# Autodesk Inventor assembly: Z assembly
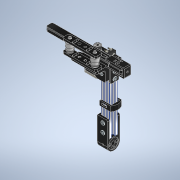
[picture p0: Inventor's stored thumbnail of the model, 180x180]
Saved by Autodesk Inventor 2022 (Build 260153000, 153)
## iProperties
Created: 2022-03-06
Part Number: Z assembly
Document SubType Name: Assembly
Designer: JK
Author: JK
## Documents named in this file (28)
- C:\Users\JK\Documents\Inventor\ScaraNema\SCARA-3DP\Parts\Forearm\Forearm assembly.iam
- C:\Users\JK\Documents\Inventor\ScaraNema\SCARA-3DP\Parts\Forearm\Z Motor support.ipt
- C:\Users\JK\Documents\Inventor\ScaraNema\SCARA-3DP\Parts\V-Slot 20x20.ipt
- C:\Users\JK\Documents\Inventor\ScaraNema\SCARA-3DP\Parts\Forearm\Z axis limit switch support.ipt
- C:\Users\JK\Documents\Inventor\ScaraNema\SCARA-3DP\Parts\Common components\V-Slot 20x20\V-Slot 20x20x150.ipt
- C:\Users\JK\Documents\Inventor\ScaraNema\SCARA-3DP\Parts\Forearm\Forearm support.ipt
- C:\Users\JK\Documents\Inventor\ScaraNema\SCARA-3DP\Parts\Common components\Limit switch.ipt
- C:\Users\JK\Documents\Inventor\ScaraNema\SCARA-3DP\Parts\Fasteners\M2x10 socket bolt.ipt
- C:\Users\JK\Documents\Inventor\ScaraNema\SCARA-3DP\Parts\Fasteners\M2 Hex nut.ipt
- C:\Users\JK\Documents\Inventor\ScaraNema\SCARA-3DP\Parts\Fasteners\M3x10 set screw.ipt
- C:\Users\JK\Documents\Inventor\ScaraNema\SCARA-3DP\Parts\Fasteners\M5x15 Flat head bolt.ipt
- C:\Users\JK\Documents\Inventor\ScaraNema\SCARA-3DP\Parts\Fasteners\M5x10 Flat head bolt.ipt
- C:\Users\JK\Documents\Inventor\ScaraNema\SCARA-3DP\Parts\Fasteners\M5x8 Flat head bolt.ipt
- C:\Users\JK\Documents\Inventor\ScaraNema\SCARA-3DP\Parts\Fasteners\M3 Hex nut.ipt
- C:\Users\JK\Documents\Inventor\ScaraNema\SCARA-3DP\Parts\Fasteners\M5 T-Nut Drop-in 20x20.ipt
- C:\Users\JK\Documents\Inventor\ScaraNema\SCARA-3DP\Parts\Fasteners\M3x6 socket bolt.ipt
- C:\Users\JK\Documents\Inventor\ScaraNema\SCARA-3DP\Parts\Forearm\yystop.ipt
- C:\Users\JK\Documents\Inventor\ScaraNema\SCARA-3DP\Parts\Forearm\Nema14 Stepper Motor v1.ipt
- C:\Users\JK\Documents\Inventor\ScaraNema\SCARA-3DP\Parts\Common components\GT2 16 Pulley.ipt
- C:\Users\JK\Documents\Inventor\ScaraNema\SCARA-3DP\Parts\Forearm\GT2RackA.ipt
- C:\Users\JK\Documents\Inventor\ScaraNema\SCARA-3DP\Parts\Forearm\tococo.ipt
- C:\Users\JK\Documents\Inventor\ScaraNema\SCARA-3DP\Parts\Forearm\GT2RackB.ipt
- C:\Users\JK\Documents\Inventor\ScaraNema\SCARA-3DP\Parts\Forearm\20T pulley 6 mm bore GT2.ipt
- C:\Users\JK\Documents\Inventor\ScaraNema\SCARA-3DP\Parts\Forearm\6mm axis.ipt
- C:\Users\JK\Documents\Inventor\ScaraNema\SCARA-3DP\Parts\Forearm\MF612.ipt
- C:\Users\JK\Documents\Inventor\ScaraNema\SCARA-3DP\Parts\Forearm\Rack support.ipt
- C:\Users\JK\Documents\Inventor\ScaraNema\SCARA-3DP\Parts\Forearm\Rack support b.ipt
- C:\Users\JK\Documents\Inventor\ScaraNema\SCARA-3DP\Parts\Forearm\magnetsupport.ipt
## Components (56 placed, 26 different names)
1. Z Motor support:1 — Coincidencia:5, Nivelación:1, Coincidencia:32, Coincidencia:48, Ángulo:19, Coincidencia:91, Coincidencia:92, Coincidencia:93, Coincidencia:94, Coincidencia:95, Coincidencia:96, Coincidencia:103, Coincidencia:104, Coincidencia:117, Tangente:2, Coincidencia:118
2. V-Slot 20x20x150:1 — Coincidencia:5, Nivelación:1, Coincidencia:16, Nivelación:8, Coincidencia:17, Coincidencia:18, Coincidencia:29, Ángulo:12, Coincidencia:97, Coincidencia:98, Coincidencia:100, Coincidencia:117
3. Z axis limit switch support:1 — Coincidencia:16, Nivelación:8, Coincidencia:20, Coincidencia:21, Coincidencia:22, Ángulo:5, Coincidencia:28, Coincidencia:29, Coincidencia:46, Coincidencia:47, Coincidencia:89, Coincidencia:90
4. Forearm support:1 — Coincidencia:17, Coincidencia:18, Coincidencia:33, Coincidencia:34, Coincidencia:35, Coincidencia:36, Coincidencia:37, Coincidencia:38, Coincidencia:42, Ángulo:8, Coincidencia:43, Coincidencia:44, Coincidencia:45, Ángulo:15, Coincidencia:83, Coincidencia:84, Coincidencia:85, Coincidencia:86, Coincidencia:88, Coincidencia:98, Coincidencia:99, Coincidencia:101, Ángulo:21
5. Limit switch:1 — Coincidencia:20, Coincidencia:21, Coincidencia:22, Coincidencia:23, Coincidencia:24, Coincidencia:25
6. M2x10 socket bolt:1 — Coincidencia:23, Nivelación:9, Coincidencia:26
7. M2x10 socket bolt:2 — Coincidencia:24, Nivelación:9, Coincidencia:25, Coincidencia:27
8. M2 Hex nut:1 — Coincidencia:27, Nivelación:10, Ángulo:4, Ángulo:5
9. M2 Hex nut:2 — Coincidencia:26, Nivelación:10, Ángulo:4, Coincidencia:28
10. M5x15 Flat head bolt:1 — Coincidencia:32, Coincidencia:73, Coincidencia:93
11. M5x10 Flat head bolt:1 — Coincidencia:33, Nivelación:12, Coincidencia:82, Coincidencia:86
12. M5x10 Flat head bolt:2 — Coincidencia:34, Nivelación:12, Coincidencia:81
13. M5x10 Flat head bolt:3 — Coincidencia:35, Nivelación:11, Coincidencia:77, Coincidencia:88
14. M5x10 Flat head bolt:4 — Coincidencia:36, Nivelación:11, Coincidencia:78
15. M5x8 Flat head bolt:1 — Coincidencia:37, Nivelación:13, Coincidencia:79, Coincidencia:99
16. M5x8 Flat head bolt:2 — Coincidencia:38, Nivelación:13, Coincidencia:80
17. M5x8 Flat head bolt:3 — Coincidencia:47, Nivelación:15, Coincidencia:75, Coincidencia:90
18. M5x8 Flat head bolt:4 — Coincidencia:46, Nivelación:15, Coincidencia:74
19. M5x15 Flat head bolt:2 — Coincidencia:48, Coincidencia:76, Coincidencia:94
20. M5 T-Nut Drop-in 20x20:1 — Coincidencia:73, Coincidencia:91
21. M5 T-Nut Drop-in 20x20:2 — Coincidencia:74, Nivelación:22, Ángulo:18, Ángulo:19
22. M5 T-Nut Drop-in 20x20:3 — Coincidencia:75, Nivelación:22, Ángulo:18, Coincidencia:89
23. M5 T-Nut Drop-in 20x20:4 — Coincidencia:76, Coincidencia:92
24. M5 T-Nut Drop-in 20x20:5 — Coincidencia:77, Ángulo:13, Nivelación:25, Ángulo:14, Ángulo:17, Coincidencia:84
25. M5 T-Nut Drop-in 20x20:6 — Coincidencia:78, Ángulo:13, Nivelación:25, Ángulo:14, Ángulo:15
26. M5 T-Nut Drop-in 20x20:7 — Coincidencia:79, Nivelación:23, Ángulo:11, Coincidencia:85
27. M5 T-Nut Drop-in 20x20:8 — Coincidencia:80, Nivelación:23, Ángulo:11, Ángulo:12
28. M5 T-Nut Drop-in 20x20:9 — Coincidencia:82, Nivelación:24, Ángulo:16, Coincidencia:83
29. M5 T-Nut Drop-in 20x20:10 — Coincidencia:81, Nivelación:24, Ángulo:16, Ángulo:17
30. yystop:1 — Coincidencia:97, Coincidencia:100, Coincidencia:101
31. Nema14 Stepper Motor v1:1 — Coincidencia:103, Coincidencia:104, Coincidencia:105, Nivelación:26
32. GT2 16 Pulley:1 — Coincidencia:105, Nivelación:26, Tangente:1, Coincidencia:116
33. GT2RackA:1 — Coincidencia:106, Ángulo:20, Coincidencia:107, Nivelación:27, Coincidencia:108, Coincidencia:109, Tangente:1, Coincidencia:116, Coincidencia:122, Ángulo:22
34. tococo:1 — Nivelación:27, Coincidencia:108, Coincidencia:109
35. GT2RackB:1 — Coincidencia:106, Ángulo:20, Coincidencia:107, Coincidencia:126, Ángulo:23, Tangente:3
36. 20T pulley 6 mm bore GT2:1 — Coincidencia:111, Nivelación:28, Coincidencia:122
37. 20T pulley 6 mm bore GT2:2 — Coincidencia:110, Nivelación:28
38. 6mm axis:1 — Coincidencia:111, Coincidencia:114, Coincidencia:115, Nivelación:29, Nivelación:32
39. 6mm axis:2 — Coincidencia:110, Coincidencia:112, Coincidencia:113, Nivelación:32, Coincidencia:125
40. MF612:1 — Coincidencia:112, Coincidencia:121, Nivelación:30
41. MF612:2 — Coincidencia:113, Nivelación:31
42. MF612:3 — Coincidencia:115, Nivelación:29, Coincidencia:119, Coincidencia:120, Nivelación:30
43. MF612:4 — Coincidencia:114, Nivelación:31, Coincidencia:123, Coincidencia:124
44. Rack support:1 — Tangente:2, Coincidencia:118, Coincidencia:119, Coincidencia:120, Ángulo:21, Coincidencia:121, Ángulo:22
45. Rack support b:1 — Coincidencia:123, Coincidencia:124, Coincidencia:125
46. magnetsupport:1 — Coincidencia:126, Ángulo:23, Tangente:3
47. M3x10 set screw:5 — Coincidencia:44, Coincidencia:45
48. M3 Hex nut:1 — Coincidencia:42, Ángulo:8, Coincidencia:43
49. M3x10 set screw:6
50. M3 Hex nut:4
51. M3x10 set screw:7
52. M3 Hex nut:5
53. M3x6 socket bolt:2 — Coincidencia:95, Coincidencia:96
54. M3x6 socket bolt:3
55. M3x6 socket bolt:4
56. M3x6 socket bolt:5
## Component patterns: (3 elements, first: M3x10 set screw:5 + M3 Hex nut:1), (4 elements, first: M3x6 socket bolt:2)
## Relationships (118: Mate 80, Flush 19, Angle 16, Tangent 3)
- Coincidencia:5 [Mate]: Z Motor support:1 ↔ V-Slot 20x20x150:1
- Nivelación:1 [Flush]: Z Motor support:1 ↔ V-Slot 20x20x150:1
- Coincidencia:16 [Mate]: V-Slot 20x20x150:1 ↔ Z axis limit switch support:1
- Nivelación:8 [Flush]: V-Slot 20x20x150:1 ↔ Z axis limit switch support:1
- Coincidencia:17 [Mate]: V-Slot 20x20x150:1 ↔ Forearm support:1
- Coincidencia:18 [Mate] (0.15 mm): V-Slot 20x20x150:1 ↔ Forearm support:1
- Coincidencia:20 [Mate]: Z axis limit switch support:1 ↔ Limit switch:1
- Coincidencia:21 [Mate]: Z axis limit switch support:1 ↔ Limit switch:1
- Coincidencia:22 [Mate]: Z axis limit switch support:1 ↔ Limit switch:1
- Coincidencia:23 [Mate]: Limit switch:1 ↔ M2x10 socket bolt:1
- Coincidencia:24 [Mate]: Limit switch:1 ↔ M2x10 socket bolt:2
- Nivelación:9 [Flush]: M2x10 socket bolt:1 ↔ M2x10 socket bolt:2
- Coincidencia:25 [Mate]: Limit switch:1 ↔ M2x10 socket bolt:2
- Coincidencia:26 [Mate]: M2x10 socket bolt:1 ↔ M2 Hex nut:2
- Coincidencia:27 [Mate]: M2x10 socket bolt:2 ↔ M2 Hex nut:1
- Nivelación:10 [Flush]: M2 Hex nut:1 ↔ M2 Hex nut:2
- Ángulo:4 [Angle] (0 deg): M2 Hex nut:1 ↔ M2 Hex nut:2
- Ángulo:5 [Angle] (0 deg): Z axis limit switch support:1 ↔ M2 Hex nut:1
- Coincidencia:28 [Mate]: Z axis limit switch support:1 ↔ M2 Hex nut:2
- Coincidencia:29 [Mate] (10 mm): V-Slot 20x20x150:1 ↔ Z axis limit switch support:1
- Coincidencia:32 [Mate]: Z Motor support:1 ↔ M5x15 Flat head bolt:1
- Coincidencia:33 [Mate]: Forearm support:1 ↔ M5x10 Flat head bolt:1
- Coincidencia:34 [Mate]: Forearm support:1 ↔ M5x10 Flat head bolt:2
- Coincidencia:35 [Mate]: Forearm support:1 ↔ M5x10 Flat head bolt:3
- Coincidencia:36 [Mate]: Forearm support:1 ↔ M5x10 Flat head bolt:4
- Nivelación:11 [Flush]: M5x10 Flat head bolt:3 ↔ M5x10 Flat head bolt:4
- Nivelación:12 [Flush]: M5x10 Flat head bolt:1 ↔ M5x10 Flat head bolt:2
- Coincidencia:37 [Mate]: Forearm support:1 ↔ M5x8 Flat head bolt:1
- Coincidencia:38 [Mate]: Forearm support:1 ↔ M5x8 Flat head bolt:2
- Nivelación:13 [Flush]: M5x8 Flat head bolt:1 ↔ M5x8 Flat head bolt:2
- Coincidencia:42 [Mate]: Forearm support:1 ↔ M3 Hex nut:1
- Ángulo:8 [Angle] (0 deg): Forearm support:1 ↔ M3 Hex nut:1
- Coincidencia:43 [Mate]: Forearm support:1 ↔ M3 Hex nut:1
- Coincidencia:44 [Mate]: Forearm support:1 ↔ M3x10 set screw:5
- Coincidencia:45 [Mate] (-5 mm): Forearm support:1 ↔ M3x10 set screw:5
- Coincidencia:46 [Mate]: Z axis limit switch support:1 ↔ M5x8 Flat head bolt:4
- Coincidencia:47 [Mate]: Z axis limit switch support:1 ↔ M5x8 Flat head bolt:3
- Nivelación:15 [Flush]: M5x8 Flat head bolt:3 ↔ M5x8 Flat head bolt:4
- Coincidencia:48 [Mate]: Z Motor support:1 ↔ M5x15 Flat head bolt:2
- Coincidencia:73 [Mate]: M5x15 Flat head bolt:1 ↔ M5 T-Nut Drop-in 20x20:1
- Coincidencia:74 [Mate]: M5x8 Flat head bolt:4 ↔ M5 T-Nut Drop-in 20x20:2
- Coincidencia:75 [Mate]: M5x8 Flat head bolt:3 ↔ M5 T-Nut Drop-in 20x20:3
- Coincidencia:76 [Mate]: M5x15 Flat head bolt:2 ↔ M5 T-Nut Drop-in 20x20:4
- Nivelación:22 [Flush]: M5 T-Nut Drop-in 20x20:2 ↔ M5 T-Nut Drop-in 20x20:3
- Coincidencia:77 [Mate]: M5x10 Flat head bolt:3 ↔ M5 T-Nut Drop-in 20x20:5
- Coincidencia:78 [Mate]: M5x10 Flat head bolt:4 ↔ M5 T-Nut Drop-in 20x20:6
- Coincidencia:79 [Mate]: M5x8 Flat head bolt:1 ↔ M5 T-Nut Drop-in 20x20:7
- Coincidencia:80 [Mate]: M5x8 Flat head bolt:2 ↔ M5 T-Nut Drop-in 20x20:8
- Coincidencia:81 [Mate]: M5x10 Flat head bolt:2 ↔ M5 T-Nut Drop-in 20x20:10
- Coincidencia:82 [Mate]: M5x10 Flat head bolt:1 ↔ M5 T-Nut Drop-in 20x20:9
- Nivelación:23 [Flush]: M5 T-Nut Drop-in 20x20:7 ↔ M5 T-Nut Drop-in 20x20:8
- Nivelación:24 [Flush]: M5 T-Nut Drop-in 20x20:9 ↔ M5 T-Nut Drop-in 20x20:10
- Ángulo:11 [Angle] (0 deg): M5 T-Nut Drop-in 20x20:7 ↔ M5 T-Nut Drop-in 20x20:8
- Ángulo:12 [Angle] (90 deg): V-Slot 20x20x150:1 ↔ M5 T-Nut Drop-in 20x20:8
- Ángulo:13 [Angle] (0 deg): M5 T-Nut Drop-in 20x20:5 ↔ M5 T-Nut Drop-in 20x20:6
- Nivelación:25 [Flush]: M5 T-Nut Drop-in 20x20:5 ↔ M5 T-Nut Drop-in 20x20:6
- Ángulo:14 [Angle] (0 deg): M5 T-Nut Drop-in 20x20:5 ↔ M5 T-Nut Drop-in 20x20:6
- Ángulo:15 [Angle] (0 deg): Forearm support:1 ↔ M5 T-Nut Drop-in 20x20:6
- Ángulo:16 [Angle] (0 deg): M5 T-Nut Drop-in 20x20:9 ↔ M5 T-Nut Drop-in 20x20:10
- Ángulo:17 [Angle] (0 deg): M5 T-Nut Drop-in 20x20:5 ↔ M5 T-Nut Drop-in 20x20:10
- Coincidencia:83 [Mate] (0.6 mm): Forearm support:1 ↔ M5 T-Nut Drop-in 20x20:9
- Coincidencia:84 [Mate] (0.6 mm): Forearm support:1 ↔ M5 T-Nut Drop-in 20x20:5
- Coincidencia:85 [Mate] (0.6 mm): Forearm support:1 ↔ M5 T-Nut Drop-in 20x20:7
- Coincidencia:86 [Mate]: Forearm support:1 ↔ M5x10 Flat head bolt:1
- Coincidencia:88 [Mate]: Forearm support:1 ↔ M5x10 Flat head bolt:3
- Ángulo:18 [Angle] (0 deg): M5 T-Nut Drop-in 20x20:2 ↔ M5 T-Nut Drop-in 20x20:3
- Ángulo:19 [Angle] (0 deg): Z Motor support:1 ↔ M5 T-Nut Drop-in 20x20:2
- Coincidencia:89 [Mate] (0.6 mm): Z axis limit switch support:1 ↔ M5 T-Nut Drop-in 20x20:3
- Coincidencia:90 [Mate]: Z axis limit switch support:1 ↔ M5x8 Flat head bolt:3
- Coincidencia:91 [Mate] (0.6 mm): Z Motor support:1 ↔ M5 T-Nut Drop-in 20x20:1
- Coincidencia:92 [Mate] (0.6 mm): Z Motor support:1 ↔ M5 T-Nut Drop-in 20x20:4
- Coincidencia:93 [Mate]: Z Motor support:1 ↔ M5x15 Flat head bolt:1
- Coincidencia:94 [Mate]: Z Motor support:1 ↔ M5x15 Flat head bolt:2
- Coincidencia:95 [Mate]: Z Motor support:1 ↔ M3x6 socket bolt:2
- Coincidencia:96 [Mate]: Z Motor support:1 ↔ M3x6 socket bolt:2
- Coincidencia:97 [Mate] (0.15 mm): V-Slot 20x20x150:1 ↔ yystop:1
- Coincidencia:98 [Mate]: V-Slot 20x20x150:1 ↔ Forearm support:1
- Coincidencia:99 [Mate]: Forearm support:1 ↔ M5x8 Flat head bolt:1
- Coincidencia:100 [Mate] (5 mm): V-Slot 20x20x150:1 ↔ yystop:1
- Coincidencia:101 [Mate] (20 mm): Forearm support:1 ↔ yystop:1
- Coincidencia:103 [Mate]: Z Motor support:1 ↔ Nema14 Stepper Motor v1:1
- Coincidencia:104 [Mate]: Z Motor support:1 ↔ Nema14 Stepper Motor v1:1
- Coincidencia:105 [Mate]: Nema14 Stepper Motor v1:1 ↔ GT2 16 Pulley:1
- Nivelación:26 [Flush]: Nema14 Stepper Motor v1:1 ↔ GT2 16 Pulley:1
- Coincidencia:106 [Mate]: GT2RackA:1 ↔ GT2RackB:1
- Ángulo:20 [Angle] (0 deg): GT2RackA:1 ↔ GT2RackB:1
- Coincidencia:107 [Mate] (1 mm): GT2RackA:1 ↔ GT2RackB:1
- Nivelación:27 [Flush]: GT2RackA:1 ↔ tococo:1
- Coincidencia:108 [Mate]: GT2RackA:1 ↔ tococo:1
- Coincidencia:109 [Mate] (0.15 mm): GT2RackA:1 ↔ tococo:1
- Coincidencia:110 [Mate]: 20T pulley 6 mm bore GT2:2 ↔ 6mm axis:2
- Coincidencia:111 [Mate]: 20T pulley 6 mm bore GT2:1 ↔ 6mm axis:1
- Nivelación:28 [Flush]: 20T pulley 6 mm bore GT2:1 ↔ 20T pulley 6 mm bore GT2:2
- Coincidencia:112 [Mate]: 6mm axis:2 ↔ MF612:1
- Coincidencia:113 [Mate]: 6mm axis:2 ↔ MF612:2
- Coincidencia:114 [Mate]: 6mm axis:1 ↔ MF612:4
- Coincidencia:115 [Mate]: 6mm axis:1 ↔ MF612:3
- Tangente:1 (-0.5 mm): GT2 16 Pulley:1 ↔ GT2RackA:1
- Coincidencia:116 [Mate] (0.5 mm): GT2 16 Pulley:1 ↔ GT2RackA:1
- Coincidencia:117 [Mate] (0.15 mm): Z Motor support:1 ↔ V-Slot 20x20x150:1
- Tangente:2: Z Motor support:1 ↔ Rack support:1
- Coincidencia:118 [Mate]: Z Motor support:1 ↔ Rack support:1
- Nivelación:29 [Flush]: 6mm axis:1 ↔ MF612:3
- Coincidencia:119 [Mate]: MF612:3 ↔ Rack support:1
- Coincidencia:120 [Mate]: MF612:3 ↔ Rack support:1
- Ángulo:21 [Angle] (0 deg): Forearm support:1 ↔ Rack support:1
- Coincidencia:121 [Mate]: MF612:1 ↔ Rack support:1
- Nivelación:30 [Flush]: MF612:1 ↔ MF612:3
- Nivelación:31 [Flush]: MF612:2 ↔ MF612:4
- Nivelación:32 [Flush]: 6mm axis:1 ↔ 6mm axis:2
- Coincidencia:122 [Mate] (0.25 mm): GT2RackA:1 ↔ 20T pulley 6 mm bore GT2:1
- Ángulo:22 [Angle] (0 deg): GT2RackA:1 ↔ Rack support:1
- Coincidencia:123 [Mate]: MF612:4 ↔ Rack support b:1
- Coincidencia:124 [Mate]: MF612:4 ↔ Rack support b:1
- Coincidencia:125 [Mate]: 6mm axis:2 ↔ Rack support b:1
- Coincidencia:126 [Mate] (0.15 mm): GT2RackB:1 ↔ magnetsupport:1
- Ángulo:23 [Angle] (0 deg): GT2RackB:1 ↔ magnetsupport:1
- Tangente:3: GT2RackB:1 ↔ magnetsupport:1
